# Autodesk Inventor assembly: Assemblage Gauche
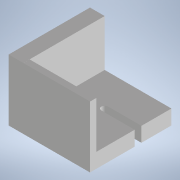
[picture p0: Inventor's stored thumbnail of the model, 180x180]
Saved by Autodesk Inventor 2020 (Build 240168000, 168)
## iProperties
Created: 2019-11-07
Part Number: Assemblage Gauche
Document SubType Name: Assembly
Designer: erwan
Author: erwan
## Documents named in this file (4)
- C:\Users\erwan\Desktop\Eirbot\Coupe robotique\Table\Support de balise\Assemblage Gauche.iam
- C:\Users\erwan\Desktop\Eirbot\Coupe robotique\Table\Support de balise\Support.ipt
- C:\Users\erwan\Desktop\Eirbot\Coupe robotique\Table\Support de balise\Fond.ipt
- C:\Users\erwan\Desktop\Eirbot\Coupe robotique\Table\Support de balise\Coté.ipt
## Components (3 placed, 3 different names)
1. Support:1 — Placage:1, Placage:2, Placage:3, Affleurement:1, Affleurement:2, Placage:4, Affleurement:3, Affleurement:4
2. Fond:1 — Placage:3, Affleurement:1, Affleurement:2
3. Coté:1 — Placage:4, Affleurement:3, Affleurement:4
## Relationships (8: Mate 4, Flush 4)
- Placage:1 [Mate]: Support:1
- Placage:2 [Mate]: Support:1
- Placage:3 [Mate]: Support:1 ↔ Fond:1
- Affleurement:1 [Flush]: Support:1 ↔ Fond:1
- Affleurement:2 [Flush]: Support:1 ↔ Fond:1
- Placage:4 [Mate]: Support:1 ↔ Coté:1
- Affleurement:3 [Flush]: Support:1 ↔ Coté:1
- Affleurement:4 [Flush]: Support:1 ↔ Coté:1
